# Autodesk Inventor assembly: OBC
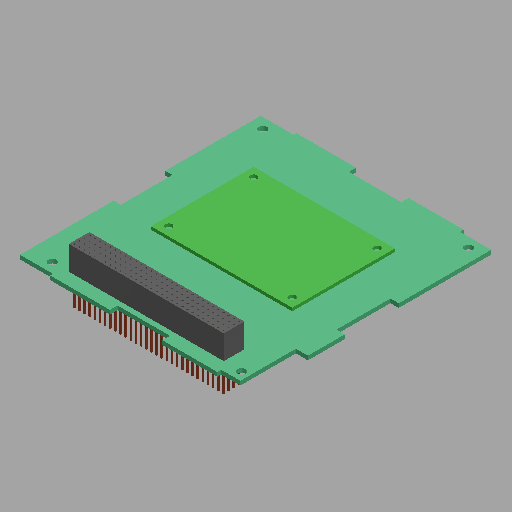
[picture p0: Inventor's stored thumbnail of the model, 512x512]
Saved by Autodesk Inventor 2022 (Build 260153000, 153)
## iProperties
Created: 2021-10-07
Part Number: OBC
Document SubType Name: Assembly
Designer: Bowen O'Steen
Author: Bowen O'Steen
## Documents named in this file (3)
- C:\Users\gwhen\OneDrive\Desktop\Vault\Designs\MEMESat\MemeSat\Engineering Data\MemeSat\Subsystems\OBC\OBC.iam
- C:\Users\gwhen\OneDrive\Desktop\Vault\Designs\MEMESat\MemeSat\Engineering Data\MemeSat\Subsystems\blankPC104plus.iam
- C:\Users\gwhen\OneDrive\Desktop\Vault\Designs\MEMESat\MemeSat\Engineering Data\MemeSat\Subsystems\OBC\rpcomputemodule4.ipt
## Components (2 placed, 2 different names)
1. blankPC104plus:1 [sub-assembly] — Mate:1, Flush:1, Flush:2, Flush:3, Flush:4, Flush:5
2. rpcomputemodule4:1 — Mate:1, Flush:1, Flush:2
## Relationships (6: Flush 5, Mate 1)
- Mate:1: blankPC104plus:1 ↔ rpcomputemodule4:1
- Flush:1 (35 mm): blankPC104plus:1 ↔ rpcomputemodule4:1
- Flush:2 (18 mm): blankPC104plus:1 ↔ rpcomputemodule4:1
- Flush:3: blankPC104plus:1
- Flush:4: blankPC104plus:1
- Flush:5: blankPC104plus:1
